# Autodesk Inventor assembly: Cover_Event_Camera_asm
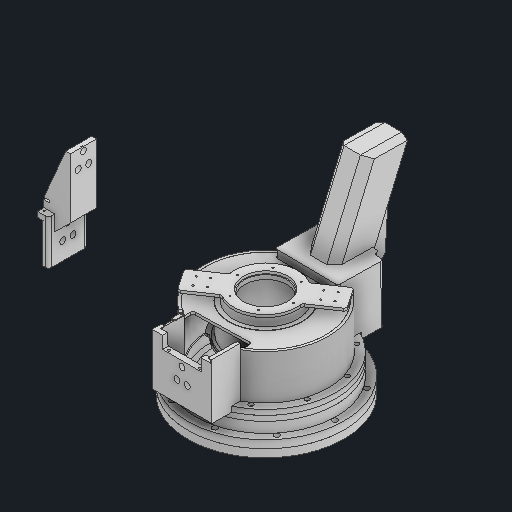
[picture p0: Inventor's stored thumbnail of the model, 512x512]
Saved by Autodesk Inventor 2026 (Build 300175000, 175)
## iProperties
Created: 2025-02-04
Part Number: Cover_Event_Camera_asm
Document SubType Name: Assembly
Designer: mayhe
Author: mayhe
## Documents named in this file (17)
- C:\School\Research\Inventor\v0.2.2\ASM\Cylinder_Cover_ASM.iam
- C:\School\Research\Inventor\v0.2.2\ASM\Cover (Optical Camera).ipt
- C:\School\Research\Inventor\v0.2.2\ASM\300mm Housing 1.ipt
- C:\School\Research\Inventor\v0.2.2\ASM\Cylinder Spacer Optical Camera.ipt
- C:\School\Research\Inventor\v0.2.2\ASM\300mm housing 2 Camera.ipt
- C:\School\Research\Inventor\v0.2.2\ASM\C .Replace - Face.ipt
- C:\School\Research\Inventor\v0.2.2\ASM\Cylinder Segment Camera Only.ipt
- C:\School\Research\Inventor\v0.2.2\ASM\C .Replace - 10.ipt
- C:\School\Research\Inventor\v0.2.2\ASM\Welding Glass.ipt
- C:\School\Research\Inventor\v0.2.2\ASM\cover^3.ipt
- C:\School\Research\Inventor\v0.2.2\ASM\Head Thing (metal).ipt
- C:\School\Research\In-situ-monitoring-of-powder-bed-fusion-additive-manufacturing\system_development\Mithril\v0.2\Model\Cover^2 No magnets.ipt
- C:\School\Research\Inventor\v0.2.2\Cover\Cover_Event_asm.iam
- C:\School\Research\Inventor\v0.2.2\ASM\Cylinder Slidey Bit Housing Both Cameras v0.1.ipt
- C:\School\Research\Inventor\v0.2.2\ASM\Cylinder Segment Both Cameras v01.ipt
- C:\School\Research\Inventor\v0.2.2\ASM\Cylinder Segment Holder Both Cameras.ipt
- C:\School\Research\Inventor\v0.2.2\ASM\Camera Bracket.ipt
## Components (15 placed, 15 different names)
1. Cover (Optical Camera):1 — Rotational:5
2. 300mm Housing 1:1 — Rotational:5, Rotational:11
3. 300mm housing 2 Camera:2 — Rotational:11, Rotational:12
4. Cylinder Spacer Optical Camera:1 — Rotational:12, Rotational:13
5. Cylinder Segment Both Cameras v01:1 — Rotational:13, Rotational:14, Rotational:15, Mate:49
6. Cylinder Slidey Bit Housing Both Cameras v0.1:1 — Rotational:14, Mate:50, Mate:51, Flush:4
7. C .Replace - Face:1 — Rotational:16, Rotational:23
8. C .Replace - 10:2 — Rotational:15, Rotational:16
9. Welding Glass:1
10. cover^3:1
11. Cylinder Segment Holder Both Cameras:1
12. Head Thing (metal):1 — Rotational:23
13. Cover^2 No magnets:1 — Mate:49
14. Cover_Event_asm:1 [sub-assembly] — Mate:50, Mate:51, Flush:4
15. Camera Bracket:1
## Relationships (14: RevoluteJoint 9, Mate 3, Flush 2)
- Rotational:5 [RevoluteJoint]: Cover (Optical Camera):1 ↔ 300mm Housing 1:1
- Rotational:11 [RevoluteJoint]: 300mm Housing 1:1 ↔ 300mm housing 2 Camera:2
- Rotational:12 [RevoluteJoint]: 300mm housing 2 Camera:2 ↔ Cylinder Spacer Optical Camera:1
- Rotational:13 [RevoluteJoint]: Cylinder Spacer Optical Camera:1 ↔ Cylinder Segment Both Cameras v01:1
- Rotational:14 [RevoluteJoint]: Cylinder Segment Both Cameras v01:1 ↔ Cylinder Slidey Bit Housing Both Cameras v0.1:1
- Rotational:15 [RevoluteJoint]: Cylinder Segment Both Cameras v01:1 ↔ C .Replace - 10:2
- Rotational:16 [RevoluteJoint]: C .Replace - Face:1 ↔ C .Replace - 10:2
- Rotational:23 [RevoluteJoint]: C .Replace - Face:1 ↔ Head Thing (metal):1
- [RevoluteJoint]: Cylinder Segment Both Cameras v01:1 ↔ Cylinder Segment Holder Both Cameras:1
- Flush:3 (128.5875 mm)
- Mate:49: Cylinder Segment Both Cameras v01:1 ↔ Cover^2 No magnets:1
- Mate:50: Cylinder Slidey Bit Housing Both Cameras v0.1:1 ↔ Cover_Event_asm:1
- Mate:51 (0.5 mm): Cylinder Slidey Bit Housing Both Cameras v0.1:1 ↔ Cover_Event_asm:1
- Flush:4: Cylinder Slidey Bit Housing Both Cameras v0.1:1 ↔ Cover_Event_asm:1
